# Autodesk Inventor assembly: catapfc1
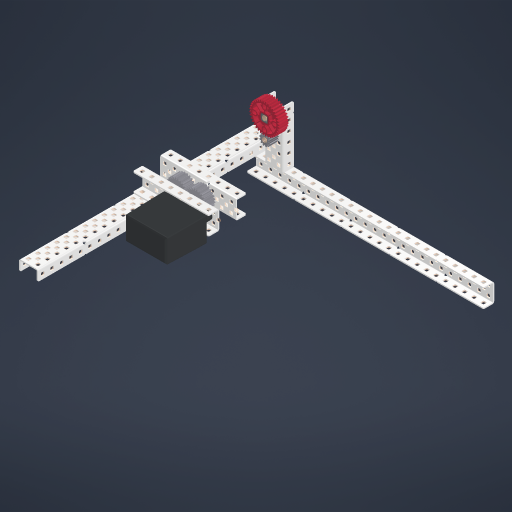
[picture p0: Inventor's stored thumbnail of the model, 512x512]
Saved by Autodesk Inventor 2024 (Build 280153000, 153)
## iProperties
Created: 2023-10-21
Part Number: catapfc1
Document SubType Name: Assembly
Designer: macbook
Author: macbook
## Documents named in this file (9)
- \\Mac\Home\Desktop\code\1599V-VRC\Cad\Assembly\v2\catapfc1.iam
- \\Mac\Home\Desktop\code\1599V-VRC\Cad\Structure\C Channel\Aluminum 1x2x1\Alu C 1x2x1x25.ipt
- \\Mac\Home\Desktop\code\1599V-VRC\Cad\Motion\Gears\HS Gear\HS 12T Gear, No Insert.iam
- \\Mac\Home\Desktop\code\1599V-VRC\Cad\Motion\Gears\HS Gear.iam
- \\Mac\Home\Desktop\code\1599V-VRC\Cad\Motion\Gears\HS Gear\HS 24T Gear, No Insert.iam
- \\Mac\Home\Desktop\code\1599V-VRC\Cad\Motion\Gears\HS Gear\HS 36T Gear, No Insert.iam
- \\Mac\Home\Desktop\code\1599V-VRC\Cad\Electronics\V5 Simple Motor.ipt
- \\Mac\Home\Desktop\code\1599V-VRC\Cad\Structure\C Channel\Aluminum 1x2x1\Alu C 1x2x1x6.ipt
- \\Mac\Home\Desktop\code\1599V-VRC\Cad\Structure\C Channel\Aluminum 1x2x1\Alu C 1x2x1x8.ipt
## Components (10 placed, 7 different names)
1. Alu C 1x2x1x25:1
2. Alu C 1x2x1x25:2 — Insert:8
3. HS 12T Gear, No Insert:1 [sub-assembly] — Insert:9
4. HS 24T Gear, No Insert:2 [sub-assembly]
5. HS 24T Gear, No Insert:3 [sub-assembly]
6. HS 36T Gear, No Insert:4 [sub-assembly] — Insert:10
7. V5 Simple Motor:1
8. Alu C 1x2x1x6:1 — Insert:8, Insert:9, Insert:10
9. Alu C 1x2x1x8:1
10. Alu C 1x2x1x8:2
## Relationships (10: Insert 10)
- [Insert] (25.4 mm): Alu C 1x2x1x25:1 ↔ Alu C 1x2x1x25:2
- [Insert] (25.4 mm): Alu C 1x2x1x25:1 ↔ Alu C 1x2x1x25:2
- [Insert]: Alu C 1x2x1x25:2 ↔ Alu C 1x2x1x8:2
- [Insert]: Alu C 1x2x1x25:2 ↔ Alu C 1x2x1x8:1
- [Insert] (6.35 mm): HS 24T Gear, No Insert:3 ↔ Alu C 1x2x1x8:1
- [Insert] (6.35 mm): HS 24T Gear, No Insert:2 ↔ Alu C 1x2x1x8:1
- [Insert]: V5 Simple Motor:1 ↔ Alu C 1x2x1x8:1
- Insert:8: Alu C 1x2x1x25:2 ↔ Alu C 1x2x1x6:1
- Insert:9: HS 12T Gear, No Insert:1 ↔ Alu C 1x2x1x6:1
- Insert:10: HS 36T Gear, No Insert:4 ↔ Alu C 1x2x1x6:1
